# Autodesk Inventor assembly: Assembly 10
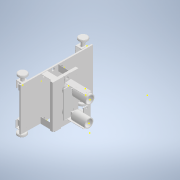
[picture p0: Inventor's stored thumbnail of the model, 180x180]
Saved by Autodesk Inventor 2020 (Build 240168000, 168)
## iProperties
Created: 2020-02-18
Part Number: Assembly 10
Document SubType Name: Assembly
Designer: Hp
Author: Hp
## Documents named in this file (14)
- C:\Users\Hp\Documents\Assembly 10.iam
- C:\Users\Hp\Documents\exp base 1.ipt
- C:\Users\Hp\Documents\expo clamp motor.ipt
- C:\Users\Hp\Documents\exp motor.ipt
- C:\Users\Hp\Documents\expo wheel.ipt
- C:\Users\Hp\Documents\clamp 2.ipt
- C:\Users\Hp\Documents\base 2.ipt
- C:\Users\Hp\Documents\dummy wheel.ipt
- C:\Users\Hp\Documents\funnel one.ipt
- C:\Users\Hp\Documents\clamp 2 pipe.ipt
- C:\Users\Hp\Documents\storage pipe 2.ipt
- C:\Users\Hp\Documents\expo clamp motor 2.ipt
- C:\Users\Hp\Documents\rack and pinion one.ipt
- C:\Users\Hp\Documents\rack and pinion 3.ipt
## Components (28 placed, 13 different names)
1. exp base 1:1 — Planar:1, Rotational:1, Planar:2, Planar:3, Planar:4, Planar:5, Planar:6, Planar:7, Planar:8, Planar:9
2. expo clamp motor:1 — Planar:5, Insert:8
3. expo clamp motor:2 — Planar:4, Insert:2, Insert:7
4. expo clamp motor:3 — Planar:2, Insert:6
5. expo clamp motor:4 — Planar:1, Rotational:1, Planar:3
6. exp motor:3
7. exp motor:4 — Insert:2
8. expo wheel:1 — Insert:8
9. expo wheel:2 — Insert:7
10. expo wheel:3 — Insert:11
11. expo wheel:4 — Insert:6
12. dummy wheel:1 — Insert:11
13. clamp 2:1 — Planar:7, Planar:10
14. clamp 2:2 — Planar:8
15. clamp 2:3 — Planar:9
16. clamp 2:4 — Planar:6
17. base 2:1 — Planar:10, Insert:12, Insert:13, Planar:11, Planar:12, Planar:13, Planar:14
18. funnel one:1 — Insert:12
19. funnel one:2 — Insert:13
20. clamp 2 pipe:1
21. clamp 2 pipe:2 — Planar:11, Planar:14, Tangent:4, Tangent:5
22. clamp 2 pipe:3 — Planar:12, Planar:13, Tangent:2, Tangent:3
23. storage pipe 2:1 — Tangent:4, Tangent:5
24. storage pipe 2:2 — Tangent:2, Tangent:3
25. expo clamp motor 2:1
26. exp motor:5
27. rack and pinion one:1
28. rack and pinion 3:1
## Relationships (27: PlanarJoint 14, Insert 7, Tangent 4, RevoluteJoint 1, Mate 1)
- Planar:1: exp base 1:1 ↔ expo clamp motor:4
- Rotational:1 [RevoluteJoint]: exp base 1:1 ↔ expo clamp motor:4
- Planar:2: exp base 1:1 ↔ expo clamp motor:3
- Planar:3: exp base 1:1 ↔ expo clamp motor:4
- Planar:4: exp base 1:1 ↔ expo clamp motor:2
- Planar:5: exp base 1:1 ↔ expo clamp motor:1
- Insert:2: expo clamp motor:2 ↔ exp motor:4
- Insert:6: expo clamp motor:3 ↔ expo wheel:4
- Insert:7: expo clamp motor:2 ↔ expo wheel:2
- Insert:8: expo clamp motor:1 ↔ expo wheel:1
- Mate:3
- Insert:11: expo wheel:3 ↔ dummy wheel:1
- Planar:6: exp base 1:1 ↔ clamp 2:4
- Planar:7: exp base 1:1 ↔ clamp 2:1
- Planar:8: exp base 1:1 ↔ clamp 2:2
- Planar:9: exp base 1:1 ↔ clamp 2:3
- Planar:10: clamp 2:1 ↔ base 2:1
- Insert:12: base 2:1 ↔ funnel one:1
- Insert:13: base 2:1 ↔ funnel one:2
- Planar:11: base 2:1 ↔ clamp 2 pipe:2
- Planar:12: base 2:1 ↔ clamp 2 pipe:3
- Planar:13: base 2:1 ↔ clamp 2 pipe:3
- Planar:14: base 2:1 ↔ clamp 2 pipe:2
- Tangent:2: clamp 2 pipe:3 ↔ storage pipe 2:2
- Tangent:3: clamp 2 pipe:3 ↔ storage pipe 2:2
- Tangent:4: clamp 2 pipe:2 ↔ storage pipe 2:1
- Tangent:5: clamp 2 pipe:2 ↔ storage pipe 2:1
